# Autodesk Inventor assembly: 305-02
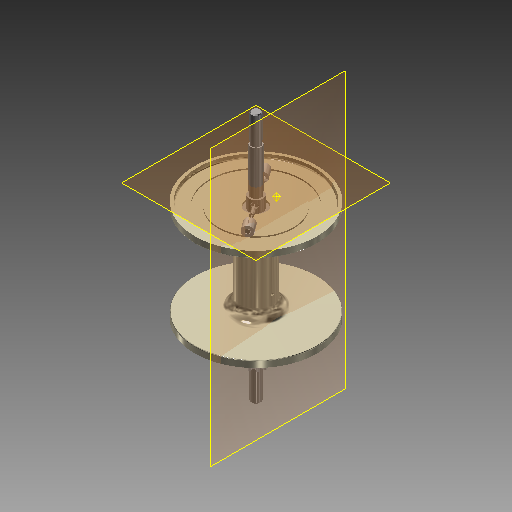
[picture p0: Inventor's stored thumbnail of the model, 512x512]
Saved by Autodesk Inventor 2019 (Build 230136000, 136)
## iProperties
Company: Autodesk Inc.
Created: 2012-01-25
Part Number: 305-02
Document SubType Name: Assembly
Designer: Autodesk Inc.
Mass: 19.2483 g
Surface Area: 92.8492 cm^2
Volume: 7.1505 cm^3
Density: 2.69188 g/cm^3
Author: Inventor
## Documents named in this file (6)
- C:\TEMP\Fishing Rod\Workspaces\Spool Assembly.iam
- C:\TEMP\Fishing Rod\Workspaces\Spool.ipt
- C:\TEMP\Fishing Rod\Workspaces\Drive Spindle Crossmember Roller.ipt
- C:\TEMP\Fishing Rod\Workspaces\Drive Spindle Crossmember.ipt
- C:\TEMP\Fishing Rod\Workspaces\Spool Drive Spindle.ipt
- C:\TEMP\Fishing Rod\Workspaces\Spool to Winder Transfer Gear.ipt
## Components (6 placed, 5 different names)
1. Spool:1 — Tangent:1, Mate:2, Flush:2
2. Drive Spindle Crossmember:1 — Insert:1, Insert:2, Mate:1, Mate:3
3. Drive Spindle Crossmember Roller:1 — Insert:1
4. Drive Spindle Crossmember Roller:2 — Insert:2, Tangent:1
5. Spool Drive Spindle:1 — Mate:1, Mate:2, Mate:3, Insert:3, Angle:1, Rotation:1
6. Spool to Winder Transfer Gear:1 — Insert:3, Angle:1, Rotation:1
## Relationships (14: Mate 6, Insert 3, Flush 2, Tangent 1, Angle 1, RelateRotation 1)
- Insert:1: Drive Spindle Crossmember:1 ↔ Drive Spindle Crossmember Roller:1
- Insert:2: Drive Spindle Crossmember:1 ↔ Drive Spindle Crossmember Roller:2
- Mate:1: Drive Spindle Crossmember:1 ↔ Spool Drive Spindle:1
- Tangent:1: Spool:1 ↔ Drive Spindle Crossmember Roller:2
- Mate:2: Spool:1 ↔ Spool Drive Spindle:1
- Mate:3: Drive Spindle Crossmember:1 ↔ Spool Drive Spindle:1
- Insert:3: Spool Drive Spindle:1 ↔ Spool to Winder Transfer Gear:1
- Angle:1 (0 deg): Spool Drive Spindle:1 ↔ Spool to Winder Transfer Gear:1
- Rotation:1 [RelateRotation] (1 ul): Spool Drive Spindle:1 ↔ Spool to Winder Transfer Gear:1
- Flush:1 (7 mm)
- Flush:2 (5 mm): Spool:1
- Mate:4
- Mate:5
- Mate:6
